# Autodesk Inventor assembly: dual_extruder
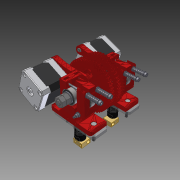
[picture p0: Inventor's stored thumbnail of the model, 180x180]
Saved by Autodesk Inventor 2014 (Build 180170000, 170)
## iProperties
Created: 2014-02-23
Part Number: dual_extruder
Document SubType Name: Assembly
Designer: buben
Author: buben
## Documents named in this file (6)
- C:\Users\buben\Documents\GitHub\bacon\inventor files\assemblies\dual_extruder.iam
- C:\Users\buben\Documents\GitHub\bacon\inventor files\assemblies\extruder.iam
- C:\Users\buben\Documents\GitHub\bacon\inventor files\assemblies\extruder_mirrored.iam
- C:\Users\buben\Documents\GitHub\bacon\inventor files\utils\hotend_mount.ipt
- C:\Users\buben\Documents\Inventor\Content Center Files\R2014\en-US\CSN EN 24017\ISO 4017 - M4 x 25CSN EN.ipt
- C:\Users\buben\Documents\GitHub\bacon\inventor files\3rd party components\j-head nozzle\Imported Components\JHead_Nozzle\JHead_Nozzle.iam
## Components (10 placed, 5 different names)
1. extruder:1 [sub-assembly] — Flush:1, Flush:2, Mate:2, Mate:3, Flush:5, Mate:8, Mate:11
2. extruder_mirrored:1 [sub-assembly] — Flush:1, Flush:2, Mate:1, Mate:9, Mate:10
3. hotend_mount:1 — Flush:3, Flush:4, Mate:6, Mate:7, Insert:2, Angle:1
4. hotend_mount:2 — Flush:3, Flush:4, Mate:1, Mate:4, Mate:5, Insert:1
5. CSN EN 24017 M4 x 25:1 — Mate:4, Flush:8, Flush:9, Angle:2
6. CSN EN 24017 M4 x 25:2 — Mate:5, Flush:9, Angle:2, Mate:9, Mate:10
7. CSN EN 24017 M4 x 25:3 — Mate:6, Flush:7, Flush:8, Angle:3
8. CSN EN 24017 M4 x 25:4 — Mate:7, Flush:7, Mate:8, Angle:3, Mate:11
9. JHead_Nozzle:1 [sub-assembly] — Insert:1, Flush:6, Mate:12
10. JHead_Nozzle:2 [sub-assembly] — Insert:2, Flush:6, Mate:12
## Relationships (26: Mate 12, Flush 9, Angle 3, Insert 2)
- Flush:1: extruder:1 ↔ extruder_mirrored:1
- Flush:2: extruder:1 ↔ extruder_mirrored:1
- Flush:3: hotend_mount:1 ↔ hotend_mount:2
- Flush:4: hotend_mount:1 ↔ hotend_mount:2
- Mate:1: extruder_mirrored:1 ↔ hotend_mount:2
- Mate:2: extruder:1
- Mate:3: extruder:1
- Flush:5: extruder:1
- Mate:4: hotend_mount:2 ↔ CSN EN 24017 M4 x 25:1
- Mate:5: hotend_mount:2 ↔ CSN EN 24017 M4 x 25:2
- Mate:6: hotend_mount:1 ↔ CSN EN 24017 M4 x 25:3
- Mate:7: hotend_mount:1 ↔ CSN EN 24017 M4 x 25:4
- Insert:1: hotend_mount:2 ↔ JHead_Nozzle:1
- Insert:2: hotend_mount:1 ↔ JHead_Nozzle:2
- Flush:6: JHead_Nozzle:1 ↔ JHead_Nozzle:2
- Angle:1 (180 deg): hotend_mount:1
- Flush:7: CSN EN 24017 M4 x 25:3 ↔ CSN EN 24017 M4 x 25:4
- Flush:8: CSN EN 24017 M4 x 25:1 ↔ CSN EN 24017 M4 x 25:3
- Flush:9: CSN EN 24017 M4 x 25:1 ↔ CSN EN 24017 M4 x 25:2
- Mate:8: extruder:1 ↔ CSN EN 24017 M4 x 25:4
- Angle:2 (0 deg): CSN EN 24017 M4 x 25:1 ↔ CSN EN 24017 M4 x 25:2
- Angle:3 (0 deg): CSN EN 24017 M4 x 25:3 ↔ CSN EN 24017 M4 x 25:4
- Mate:9: extruder_mirrored:1 ↔ CSN EN 24017 M4 x 25:2
- Mate:10: extruder_mirrored:1 ↔ CSN EN 24017 M4 x 25:2
- Mate:11: extruder:1 ↔ CSN EN 24017 M4 x 25:4
- Mate:12 (65 mm): JHead_Nozzle:1 ↔ JHead_Nozzle:2
